# Autodesk Inventor assembly: Additional_Building
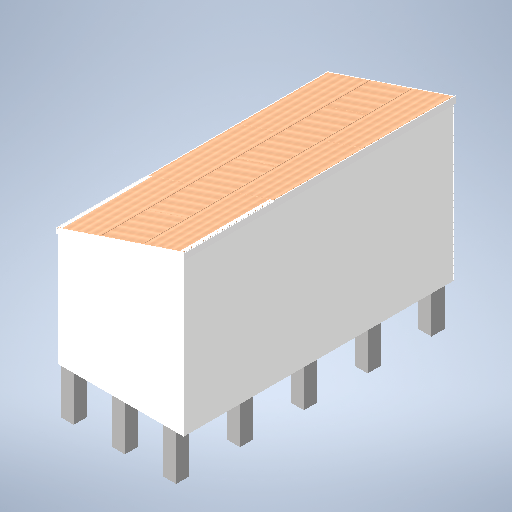
[picture p0: Inventor's stored thumbnail of the model, 512x512]
Saved by Autodesk Inventor 2025.1 (Build 291241020, 241B)
## iProperties
Created: 2024-08-02
Part Number: Additional_Building
Document SubType Name: Assembly
Designer: Tom
Author: Tom
## Documents named in this file (49)
- C:\Users\Tom\Documents\Inventor\Mobility\Additional_Building\Additional_Building.iam
- C:\Users\Tom\Documents\Inventor\Mobility\Additional_Building\Grid_Of_Piers.iam
- C:\Users\Tom\Documents\Inventor\Mobility\Additional_Building\Floor_System.iam
- C:\Users\Tom\Documents\Inventor\Mobility\Additional_Building\Walls.iam
- C:\Users\Tom\Documents\Inventor\Mobility\Additional_Building\Truss.iam
- C:\Users\Tom\Documents\Inventor\Mobility\Additional_Building\OSB_For_Walls_With_Dimensions_48_x_96_Inches.ipt
- C:\Users\Tom\Documents\Inventor\Mobility\Additional_Building\OSB_For_Walls_With_Dimensions_48_x_48_Inches.ipt
- C:\Users\Tom\Documents\Inventor\Mobility\Additional_Building\OSB_For_Roof_With_Dimensions_96_x_48.ipt
- C:\Users\Tom\Documents\Inventor\Mobility\Additional_Building\OSB_For_Walls_With_Dimensions_25.5_x_96_Inches.ipt
- C:\Users\Tom\Documents\Inventor\Mobility\Additional_Building\Subfascia_With_Dimensions_4.023_x_13.75_Inches.ipt
- C:\Users\Tom\Documents\Inventor\Mobility\Additional_Building\Subfascia_With_Dimensions_4.023_x_14.5_Inches.ipt
- C:\Users\Tom\Documents\Inventor\Mobility\Additional_Building\DensGlass_With_Dimensions_36.5_x_48_Inches.ipt
- C:\Users\Tom\Documents\Inventor\Mobility\Additional_Building\DensGlass_With_Dimensions_48_x_96_Inches.ipt
- C:\Users\Tom\Documents\Inventor\Mobility\Additional_Building\DensGlass_With_Dimensions_48_x_84.5_Inches.ipt
- C:\Users\Tom\Documents\Inventor\Mobility\Additional_Building\DensGlass_With_Dimensions_60.75_x_12_Inches.ipt
- C:\Users\Tom\Documents\Inventor\Mobility\Additional_Building\DensGlass_With_Dimensions_36.5_x_25.5_Inches.ipt
- C:\Users\Tom\Documents\Inventor\Mobility\Additional_Building\DensGlass_With_Dimensions_25.5_x_96_Inches.ipt
- C:\Users\Tom\Documents\Inventor\Mobility\Additional_Building\Siding_For_Back_Wall.iam
- C:\Users\Tom\Documents\Inventor\Mobility\Additional_Building\Fascia_For_Back.ipt
- C:\Users\Tom\Documents\Inventor\Mobility\Additional_Building\OSB_For_Side_And_Back.ipt
- C:\Users\Tom\Documents\Inventor\Mobility\Additional_Building\OSB_For_Roof_With_Dimensions_48_x_48.ipt
- C:\Users\Tom\Documents\Inventor\Mobility\Additional_Building\OSB_For_Roof_With_Dimensions_46.791_x_96.ipt
- C:\Users\Tom\Documents\Inventor\Mobility\Additional_Building\Stud_Between_Top_Plate_And_Rafter_1.ipt
- C:\Users\Tom\Documents\Inventor\Mobility\Additional_Building\Stud_Between_Top_Plate_And_Rafter_2.ipt
- C:\Users\Tom\Documents\Inventor\Mobility\Additional_Building\Stud_Between_Top_Plate_And_Rafter_3.ipt
- C:\Users\Tom\Documents\Inventor\Mobility\Additional_Building\Stud_Between_Top_Plate_And_Rafter_4.ipt
- C:\Users\Tom\Documents\Inventor\Mobility\Additional_Building\Stud_Between_Top_Plate_And_Rafter_5.ipt
- C:\Users\Tom\Documents\Inventor\Mobility\Additional_Building\Stud_Between_Top_Plate_And_Rafter_6.ipt
- C:\Users\Tom\Documents\Inventor\Mobility\Additional_Building\Stud_Between_Top_Plate_And_Rafter_7.ipt
- C:\Users\Tom\Documents\Inventor\Mobility\Additional_Building\Stud_Between_Top_Plate_And_Rafter_8.ipt
- C:\Users\Tom\Documents\Inventor\Mobility\Additional_Building\Stud_Between_Top_Plate_And_Rafter_9.ipt
- C:\Users\Tom\Documents\Inventor\Mobility\Additional_Building\Stud_With_Height_41.707_Inches.ipt
- C:\Users\Tom\Documents\Inventor\Mobility\Additional_Building\Support_For_Ceiling.ipt
- C:\Users\Tom\Documents\Inventor\Mobility\Additional_Building\OSB_For_Side_And_Front.ipt
- C:\Users\Tom\Documents\Inventor\Mobility\Additional_Building\OSB_For_Side_And_Top.ipt
- C:\Users\Tom\Documents\Inventor\Mobility\Additional_Building\Subfascia_With_Dimensions_5.798_x_13.75_Inches.ipt
- C:\Users\Tom\Documents\Inventor\Mobility\Additional_Building\Subfascia_With_Dimensions_5.798_x_14.5_Inches.ipt
- C:\Users\Tom\Documents\Inventor\Mobility\Additional_Building\OSB_For_Walls_With_Dimensions_20.604_x_48_Inches.ipt
- C:\Users\Tom\Documents\Inventor\Mobility\Additional_Building\OSB_For_Walls_With_Dimensions_20.604_x_96_Inches.ipt
- C:\Users\Tom\Documents\Inventor\Mobility\Additional_Building\Siding_For_Front_Wall.iam
- C:\Users\Tom\Documents\Inventor\Mobility\Additional_Building\Fascia_For_Front.ipt
- C:\Users\Tom\Documents\Inventor\Mobility\Additional_Building\OSB_For_Walls_With_Dimensions_48_x_85_Inches.ipt
- C:\Users\Tom\Documents\Inventor\Mobility\Additional_Building\OSB_For_Walls_With_Dimensions_37_x_48_Inches.ipt
- C:\Users\Tom\Documents\Inventor\Mobility\Additional_Building\Fascia_For_Side.ipt
- C:\Users\Tom\Documents\Inventor\Mobility\Additional_Building\Drip_Edge_For_Back.ipt
- C:\Users\Tom\Documents\Inventor\Mobility\Additional_Building\OSB_For_Rear_Roof.ipt
- C:\Users\Tom\Documents\Inventor\Mobility\Additional_Building\Siding_For_Left_Wall.iam
- C:\Users\Tom\Documents\Inventor\Mobility\Additional_Building\Siding_For_Right_Wall.iam
- C:\Users\Tom\Documents\Inventor\Mobility\Additional_Building\Drip_Edge_For_Front.ipt
## Components (175 placed, 48 different names)
1. Grid_Of_Piers:1 [sub-assembly] — Mate:1, Flush:1, Mate:2
2. Floor_System:1 [sub-assembly] — Mate:1, Flush:1, Mate:2, Mate:3, Flush:2, Flush:3, Flush:15, Flush:16, Flush:29, Flush:30, Flush:31, Flush:33
3. Walls:1 [sub-assembly] — Mate:3, Flush:2, Flush:3, Flush:4, Flush:5, Mate:4, Flush:7, Mate:5, Mate:9, Mate:10, Flush:17, Mate:12, Mate:15, Mate:18, Mate:68, Flush:48, Flush:49, Mate:69, Flush:50, Flush:51, Mate:70, Flush:52, Flush:53, Mate:71, Flush:54, Flush:55, Mate:72, Flush:56, Flush:57, Mate:73, Flush:58, Flush:59, Mate:74, Flush:60, Flush:61, Mate:75, Flush:62, Flush:63, Mate:76, Flush:64, Mate:78, Mate:90, Mate:113, Mate:116, Mate:119, Mate:121
4. Subfascia_With_Dimensions_4.023_x_13.75_Inches:1 — Mate:21, Flush:22, Flush:23
5. Subfascia_With_Dimensions_4.023_x_13.75_Inches:2 — Flush:26, Mate:23, Flush:27, Flush:39
6. DensGlass_With_Dimensions_36.5_x_48_Inches:1 — Mate:24, Flush:28, Flush:29, Mate:26
7. DensGlass_With_Dimensions_36.5_x_48_Inches:2 — Mate:27, Mate:28, Flush:31
8. DensGlass_With_Dimensions_48_x_84.5_Inches:1 — Mate:29, Flush:32, Mate:30, Mate:32, Mate:38, Mate:41, Mate:44
9. DensGlass_With_Dimensions_48_x_96_Inches:3 — Mate:31, Mate:32, Mate:33, Mate:35
10. DensGlass_With_Dimensions_48_x_84.5_Inches:2 — Mate:34, Mate:35, Mate:36, Mate:47
11. DensGlass_With_Dimensions_36.5_x_25.5_Inches:1 — Mate:39, Mate:40, Mate:41, Mate:43
12. DensGlass_With_Dimensions_36.5_x_25.5_Inches:2 — Mate:45, Mate:46, Mate:47
13. Siding_For_Back_Wall:1 [sub-assembly] — Mate:48, Flush:34, Flush:35
14. Siding_For_Front_Wall:1 [sub-assembly] — Flush:93, Flush:94, Mate:108
15. Fascia_For_Side:1 — Mate:126, Flush:103, Flush:105, Flush:108
16. Fascia_For_Side:2 — Mate:127, Flush:107, Flush:108
17. Drip_Edge_For_Back:1 — Flush:109, Mate:128, Mate:137
18. Siding_For_Left_Wall:1 [sub-assembly] — Mate:133, Flush:117, Mate:134
19. Siding_For_Right_Wall:1 [sub-assembly] — Mate:135, Mate:136, Flush:118
20. Drip_Edge_For_Front:1 — Mate:138, Flush:119, Mate:139
21. Truss:1 [sub-assembly] — Flush:6, Mate:23, Flush:27, Mate:50, Mate:56, Mate:77, Mate:79, Flush:65, Flush:67, Flush:69, Flush:71, Flush:73, Flush:75, Flush:77, Flush:79, Flush:81, Mate:92, Mate:96, Mate:109, Flush:103, Flush:104, Flush:115, Mate:132, Flush:116
22. Truss:2 [sub-assembly] — Flush:4, Flush:5, Mate:4, Mate:20, Mate:62, Mate:66, Mate:101, Flush:91, Mate:103, Flush:92
23. Truss:3 [sub-assembly] — Flush:6, Flush:7, Mate:5, Flush:26, Mate:81, Mate:82, Mate:83, Mate:84, Mate:85, Mate:86, Mate:87, Mate:88, Mate:89, Mate:91, Flush:82, Mate:99, Flush:87, Flush:88
24. Truss:4 [sub-assembly] — Mate:100, Flush:89, Flush:90
25. Truss:5 [sub-assembly]
26. Truss:6 [sub-assembly]
27. Truss:7 [sub-assembly]
28. Truss:8 [sub-assembly]
29. Truss:9 [sub-assembly]
30. Truss:10 [sub-assembly]
31. Truss:11 [sub-assembly]
32. Truss:12 [sub-assembly]
33. Truss:13 [sub-assembly]
34. Truss:14 [sub-assembly]
35. Truss:15 [sub-assembly] — Mate:63
36. Truss:16 [sub-assembly] — Mate:105
37. Truss:17 [sub-assembly]
38. Truss:18 [sub-assembly] — Mate:22, Flush:25
39. Truss:19 [sub-assembly] — Mate:21, Flush:22, Flush:23, Flush:24
40. OSB_For_Roof_With_Dimensions_96_x_48:4 — Mate:63, Mate:65
41. OSB_For_Roof_With_Dimensions_96_x_48:5
42. Subfascia_With_Dimensions_4.023_x_14.5_Inches:1 — Flush:24, Mate:22, Flush:25
43. Subfascia_With_Dimensions_4.023_x_14.5_Inches:2
44. Subfascia_With_Dimensions_4.023_x_14.5_Inches:3
45. Subfascia_With_Dimensions_4.023_x_14.5_Inches:4
46. Subfascia_With_Dimensions_4.023_x_14.5_Inches:5
47. Subfascia_With_Dimensions_4.023_x_14.5_Inches:6
48. Subfascia_With_Dimensions_4.023_x_14.5_Inches:7
49. Subfascia_With_Dimensions_4.023_x_14.5_Inches:8
50. Subfascia_With_Dimensions_4.023_x_14.5_Inches:9
51. Subfascia_With_Dimensions_4.023_x_14.5_Inches:10
52. Subfascia_With_Dimensions_4.023_x_14.5_Inches:11
53. Subfascia_With_Dimensions_4.023_x_14.5_Inches:12
54. Subfascia_With_Dimensions_4.023_x_14.5_Inches:13
55. Subfascia_With_Dimensions_4.023_x_14.5_Inches:14
56. Subfascia_With_Dimensions_4.023_x_14.5_Inches:15
57. Subfascia_With_Dimensions_4.023_x_14.5_Inches:16
58. DensGlass_With_Dimensions_48_x_96_Inches:1 — Mate:25, Mate:26, Flush:30, Mate:30, Mate:33
59. DensGlass_With_Dimensions_48_x_96_Inches:2 — Mate:28, Mate:36
60. DensGlass_With_Dimensions_60.75_x_12_Inches:1 — Mate:37, Mate:38, Flush:33
61. DensGlass_With_Dimensions_60.75_x_12_Inches:2 — Mate:48, Flush:34, Flush:35
62. DensGlass_With_Dimensions_60.75_x_12_Inches:3 — Mate:40
63. DensGlass_With_Dimensions_60.75_x_12_Inches:4 — Mate:57, Mate:115
64. DensGlass_With_Dimensions_25.5_x_96_Inches:1 — Mate:42, Mate:43, Mate:44
65. DensGlass_With_Dimensions_25.5_x_96_Inches:2 — Mate:46
66. Stud_Between_Top_Plate_And_Rafter_1:1 — Mate:68, Flush:48, Flush:49, Flush:66
67. Stud_Between_Top_Plate_And_Rafter_2:1 — Mate:69, Flush:50, Flush:51, Flush:68
68. Stud_Between_Top_Plate_And_Rafter_3:1 — Mate:70, Flush:52, Flush:53, Flush:70
69. Stud_Between_Top_Plate_And_Rafter_4:1 — Mate:71, Flush:54, Flush:55, Flush:72
70. Stud_Between_Top_Plate_And_Rafter_5:1 — Mate:72, Flush:56, Flush:57, Flush:74
71. Stud_Between_Top_Plate_And_Rafter_6:1 — Mate:73, Flush:58, Flush:59, Flush:76
72. Stud_Between_Top_Plate_And_Rafter_7:1 — Mate:74, Flush:60, Flush:61, Flush:78
73. Stud_Between_Top_Plate_And_Rafter_9:1 — Mate:76, Mate:77, Flush:64, Mate:80
74. Stud_Between_Top_Plate_And_Rafter_8:1 — Mate:75, Flush:62, Flush:63, Flush:80
75. Stud_Between_Top_Plate_And_Rafter_1:2
76. Stud_Between_Top_Plate_And_Rafter_2:2
77. Stud_Between_Top_Plate_And_Rafter_3:2
78. Stud_Between_Top_Plate_And_Rafter_4:2
79. Stud_Between_Top_Plate_And_Rafter_5:2
80. Stud_Between_Top_Plate_And_Rafter_6:2
81. Stud_Between_Top_Plate_And_Rafter_7:2
82. Stud_Between_Top_Plate_And_Rafter_9:2
83. Stud_Between_Top_Plate_And_Rafter_8:2
84. Stud_With_Height_41.707_Inches:1 — Mate:78, Mate:79, Mate:80
85. Stud_With_Height_41.707_Inches:2
86. Support_For_Ceiling:9 — Mate:89, Flush:81, Mate:90
87. Support_For_Ceiling:1 — Mate:81, Flush:65, Flush:66
88. Support_For_Ceiling:2 — Mate:82, Flush:67, Flush:68
89. Support_For_Ceiling:3 — Mate:83, Flush:69, Flush:70
90. Support_For_Ceiling:4 — Mate:84, Flush:71, Flush:72
91. Support_For_Ceiling:5 — Mate:85, Flush:73, Flush:74
92. Support_For_Ceiling:6 — Mate:86, Flush:75, Flush:76
93. Support_For_Ceiling:7 — Mate:87, Flush:77, Flush:78
94. Support_For_Ceiling:8 — Mate:88, Flush:79, Flush:80
95. Support_For_Ceiling:10 — Mate:91, Flush:82, Mate:92
96. Support_For_Ceiling:11
97. Support_For_Ceiling:12
98. Support_For_Ceiling:13
99. Support_For_Ceiling:14
100. Support_For_Ceiling:15
101. Support_For_Ceiling:16
102. Support_For_Ceiling:17
103. Support_For_Ceiling:18
104. Support_For_Ceiling:19
105. Support_For_Ceiling:20
106. Subfascia_With_Dimensions_5.798_x_13.75_Inches:1 — Mate:99, Flush:87, Flush:88
107. Subfascia_With_Dimensions_5.798_x_13.75_Inches:2
108. Subfascia_With_Dimensions_5.798_x_14.5_Inches:1 — Mate:100, Flush:89, Flush:90
109. Subfascia_With_Dimensions_5.798_x_14.5_Inches:2
110. Subfascia_With_Dimensions_5.798_x_14.5_Inches:3
111. Subfascia_With_Dimensions_5.798_x_14.5_Inches:4
112. Subfascia_With_Dimensions_5.798_x_14.5_Inches:5
113. Subfascia_With_Dimensions_5.798_x_14.5_Inches:6
114. Subfascia_With_Dimensions_5.798_x_14.5_Inches:7
115. Subfascia_With_Dimensions_5.798_x_14.5_Inches:8
116. Subfascia_With_Dimensions_5.798_x_14.5_Inches:9
117. Subfascia_With_Dimensions_5.798_x_14.5_Inches:10
118. Subfascia_With_Dimensions_5.798_x_14.5_Inches:11
119. Subfascia_With_Dimensions_5.798_x_14.5_Inches:12
120. Subfascia_With_Dimensions_5.798_x_14.5_Inches:13
121. Subfascia_With_Dimensions_5.798_x_14.5_Inches:14
122. Subfascia_With_Dimensions_5.798_x_14.5_Inches:15
123. Subfascia_With_Dimensions_5.798_x_14.5_Inches:16
124. OSB_For_Walls_With_Dimensions_25.5_x_96_Inches:1 — Mate:18, Flush:18, Mate:20, Mate:39
125. OSB_For_Walls_With_Dimensions_25.5_x_96_Inches:2 — Mate:42
126. OSB_For_Walls_With_Dimensions_25.5_x_96_Inches:3 — Mate:45
127. OSB_For_Walls_With_Dimensions_48_x_48_Inches:2 — Mate:15, Mate:16, Mate:17, Mate:29, Flush:32
128. OSB_For_Walls_With_Dimensions_48_x_48_Inches:1 — Mate:10, Mate:11, Flush:17, Mate:13, Mate:34
129. OSB_For_Walls_With_Dimensions_48_x_48_Inches:3 — Mate:102
130. OSB_For_Walls_With_Dimensions_48_x_48_Inches:4
131. OSB_For_Walls_With_Dimensions_48_x_96_Inches:13 — Mate:101, Mate:102, Flush:91, Mate:104, Mate:108
132. OSB_For_Walls_With_Dimensions_48_x_96_Inches:14 — Mate:106
133. OSB_For_Walls_With_Dimensions_48_x_96_Inches:15
134. OSB_For_Walls_With_Dimensions_20.604_x_96_Inches:1 — Mate:105, Mate:106, Mate:107
135. OSB_For_Walls_With_Dimensions_20.604_x_96_Inches:2
136. OSB_For_Walls_With_Dimensions_20.604_x_48_Inches:1 — Mate:103, Mate:104, Flush:92, Mate:107
137. OSB_For_Walls_With_Dimensions_20.604_x_48_Inches:2
138. Fascia_For_Back:1 — Mate:50, Flush:39, Flush:104, Flush:105, Flush:109, Mate:128, Mate:134
139. Fascia_For_Back:2
140. Fascia_For_Back:3 — Mate:136
141. Fascia_For_Front:1 — Mate:109, Flush:95, Flush:96, Mate:126, Mate:138, Flush:119
142. Fascia_For_Front:2
143. Fascia_For_Front:3 — Mate:127, Flush:107
144. OSB_For_Walls_With_Dimensions_48_x_96_Inches:16 — Mate:119, Mate:120, Flush:98, Mate:131, Mate:133, Flush:117
145. OSB_For_Walls_With_Dimensions_37_x_48_Inches:1 — Mate:121, Mate:122, Mate:131
146. OSB_For_Walls_With_Dimensions_48_x_48_Inches:5 — Mate:113, Mate:114, Mate:115, Mate:117, Mate:120
147. OSB_For_Walls_With_Dimensions_48_x_85_Inches:1 — Mate:116, Mate:117, Mate:118, Mate:122
148. OSB_For_Side_And_Back:1 — Mate:56, Mate:57, Flush:83, Mate:98, Mate:111, Mate:112, Mate:114, Mate:118
149. OSB_For_Side_And_Front:1 — Flush:83, Mate:97, Mate:111, Mate:112, Flush:97
150. OSB_For_Side_And_Top:1 — Mate:96, Mate:97, Flush:95, Flush:96, Flush:97, Flush:114
151. OSB_For_Walls_With_Dimensions_48_x_96_Inches:17 — Mate:135
152. OSB_For_Walls_With_Dimensions_37_x_48_Inches:2 — Flush:118
153. OSB_For_Walls_With_Dimensions_48_x_48_Inches:6
154. OSB_For_Walls_With_Dimensions_48_x_85_Inches:2
155. OSB_For_Side_And_Back:2
156. OSB_For_Side_And_Front:2
157. OSB_For_Side_And_Top:2
158. OSB_For_Roof_With_Dimensions_46.791_x_96:1 — Mate:66, Mate:67, Flush:47
159. OSB_For_Roof_With_Dimensions_46.791_x_96:2
160. OSB_For_Roof_With_Dimensions_46.791_x_96:3 — Flush:114, Mate:139
161. OSB_For_Rear_Roof:1 — Flush:115, Mate:132, Flush:116
162. OSB_For_Rear_Roof:2 — Mate:137
163. OSB_For_Rear_Roof:3
164. OSB_For_Roof_With_Dimensions_48_x_48:1 — Mate:62, Mate:65, Mate:67, Flush:47
165. OSB_For_Roof_With_Dimensions_48_x_48:2
166. OSB_For_Walls_With_Dimensions_48_x_96_Inches:1 — Mate:9, Flush:15, Flush:16, Mate:11, Mate:16, Flush:18, Mate:24, Flush:28, Mate:25, Mate:37
167. OSB_For_Walls_With_Dimensions_48_x_96_Inches:2
168. OSB_For_Walls_With_Dimensions_48_x_96_Inches:3 — Mate:14, Mate:27, Flush:98
169. OSB_For_Walls_With_Dimensions_48_x_96_Inches:4 — Mate:12, Mate:13, Mate:14, Mate:31
170. OSB_For_Walls_With_Dimensions_48_x_96_Inches:5 — Mate:17
171. OSB_For_Walls_With_Dimensions_48_x_96_Inches:8 — Flush:93, Flush:94
172. OSB_For_Walls_With_Dimensions_48_x_96_Inches:9
173. OSB_For_Walls_With_Dimensions_48_x_96_Inches:10
174. OSB_For_Walls_With_Dimensions_48_x_96_Inches:11
175. OSB_For_Walls_With_Dimensions_48_x_96_Inches:12
## Component patterns: (2 elements, first: Truss:1), (17 elements, first: Truss:3), (2 elements, first: OSB_For_Roof_With_Dimensions_96_x_48:4), (16 elements, first: Subfascia_With_Dimensions_4.023_x_14.5_Inches:1), (2 elements, first: DensGlass_With_Dimensions_48_x_96_Inches:1), (4 elements, first: DensGlass_With_Dimensions_60.75_x_12_Inches:1), (2 elements, first: DensGlass_With_Dimensions_25.5_x_96_Inches:1), (2 elements, first: Stud_Between_Top_Plate_And_Rafter_1:1 + Stud_Between_Top_Plate_And_Rafter_2:1 + Stud_Between_Top_Plate_And_Rafter_3:1 + Stud_Between_Top_Plate_And_Rafter_4:1 + Stud_Between_Top_Plate_And_Rafter_5:1 + Stud_Between_Top_Plate_And_Rafter_6:1 + Stud_Between_Top_Plate_And_Rafter_7:1 + Stud_Between_Top_Plate_And_Rafter_9:1 + Stud_Between_Top_Plate_And_Rafter_8:1), (2 elements, first: Stud_With_Height_41.707_Inches:1), (2 elements, first: Support_For_Ceiling:9 + Support_For_Ceiling:1 + Support_For_Ceiling:2 + Support_For_Ceiling:3 + Support_For_Ceiling:4 + Support_For_Ceiling:5 + Support_For_Ceiling:6 + Support_For_Ceiling:7 + Support_For_Ceiling:8 + Support_For_Ceiling:10), (2 elements, first: Subfascia_With_Dimensions_5.798_x_13.75_Inches:1), (16 elements, first: Subfascia_With_Dimensions_5.798_x_14.5_Inches:1), (3 elements, first: OSB_For_Walls_With_Dimensions_25.5_x_96_Inches:1), (2 elements, first: OSB_For_Walls_With_Dimensions_48_x_48_Inches:2 + OSB_For_Walls_With_Dimensions_48_x_48_Inches:1), (3 elements, first: OSB_For_Walls_With_Dimensions_48_x_96_Inches:13), (2 elements, first: OSB_For_Walls_With_Dimensions_20.604_x_96_Inches:1), (2 elements, first: OSB_For_Walls_With_Dimensions_20.604_x_48_Inches:1), (3 elements, first: Fascia_For_Back:1), (3 elements, first: Fascia_For_Front:1), (2 elements, first: OSB_For_Walls_With_Dimensions_48_x_96_Inches:16 + OSB_For_Walls_With_Dimensions_37_x_48_Inches:1 + OSB_For_Walls_With_Dimensions_48_x_48_Inches:5 + OSB_For_Walls_With_Dimensions_48_x_85_Inches:1 + OSB_For_Side_And_Back:1 + OSB_For_Side_And_Front:1 + OSB_For_Side_And_Top:1), (3 elements, first: OSB_For_Roof_With_Dimensions_46.791_x_96:1), (3 elements, first: OSB_For_Rear_Roof:1), (2 elements, first: OSB_For_Roof_With_Dimensions_48_x_48:1), (3 elements, first: OSB_For_Walls_With_Dimensions_48_x_96_Inches:1), (2 elements, first: OSB_For_Walls_With_Dimensions_48_x_96_Inches:4), Component Pattern 3:2 (3 elements), Component Pattern 4:2 (2 elements)
## Relationships (203: Mate 115, Flush 87, Angle 1)
- Mate:1: Grid_Of_Piers:1 ↔ Floor_System:1
- Flush:1: Grid_Of_Piers:1 ↔ Floor_System:1
- Mate:2: Grid_Of_Piers:1 ↔ Floor_System:1
- Mate:3: Floor_System:1 ↔ Walls:1
- Flush:2: Floor_System:1 ↔ Walls:1
- Flush:3: Floor_System:1 ↔ Walls:1
- Flush:4: Walls:1 ↔ Truss:2
- Flush:5: Walls:1 ↔ Truss:2
- Mate:4: Walls:1 ↔ Truss:2
- Flush:6 (387.35 mm): Truss:1 ↔ Truss:3
- Flush:7: Walls:1 ↔ Truss:3
- Mate:5: Walls:1 ↔ Truss:3
- Mate:9: Walls:1 ↔ OSB_For_Walls_With_Dimensions_48_x_96_Inches:1
- Flush:15: Floor_System:1 ↔ OSB_For_Walls_With_Dimensions_48_x_96_Inches:1
- Flush:16: Floor_System:1 ↔ OSB_For_Walls_With_Dimensions_48_x_96_Inches:1
- Mate:10: Walls:1 ↔ OSB_For_Walls_With_Dimensions_48_x_48_Inches:1
- Mate:11: OSB_For_Walls_With_Dimensions_48_x_48_Inches:1 ↔ OSB_For_Walls_With_Dimensions_48_x_96_Inches:1
- Flush:17: Walls:1 ↔ OSB_For_Walls_With_Dimensions_48_x_48_Inches:1
- Mate:12: Walls:1 ↔ OSB_For_Walls_With_Dimensions_48_x_96_Inches:4
- Mate:13: OSB_For_Walls_With_Dimensions_48_x_48_Inches:1 ↔ OSB_For_Walls_With_Dimensions_48_x_96_Inches:4
- Mate:14: OSB_For_Walls_With_Dimensions_48_x_96_Inches:3 ↔ OSB_For_Walls_With_Dimensions_48_x_96_Inches:4
- Mate:15: Walls:1 ↔ OSB_For_Walls_With_Dimensions_48_x_48_Inches:2
- Mate:16: OSB_For_Walls_With_Dimensions_48_x_48_Inches:2 ↔ OSB_For_Walls_With_Dimensions_48_x_96_Inches:1
- Mate:17: OSB_For_Walls_With_Dimensions_48_x_48_Inches:2 ↔ OSB_For_Walls_With_Dimensions_48_x_96_Inches:5
- Mate:18: Walls:1 ↔ OSB_For_Walls_With_Dimensions_25.5_x_96_Inches:1
- Flush:18: OSB_For_Walls_With_Dimensions_25.5_x_96_Inches:1 ↔ OSB_For_Walls_With_Dimensions_48_x_96_Inches:1
- Mate:20: Truss:2 ↔ OSB_For_Walls_With_Dimensions_25.5_x_96_Inches:1
- Mate:21: Subfascia_With_Dimensions_4.023_x_13.75_Inches:1 ↔ Truss:19
- Flush:22: Subfascia_With_Dimensions_4.023_x_13.75_Inches:1 ↔ Truss:19
- Flush:23: Subfascia_With_Dimensions_4.023_x_13.75_Inches:1 ↔ Truss:19
- Flush:24: Truss:19 ↔ Subfascia_With_Dimensions_4.023_x_14.5_Inches:1
- Mate:22: Truss:18 ↔ Subfascia_With_Dimensions_4.023_x_14.5_Inches:1
- Flush:25: Truss:18 ↔ Subfascia_With_Dimensions_4.023_x_14.5_Inches:1
- Flush:26: Subfascia_With_Dimensions_4.023_x_13.75_Inches:2 ↔ Truss:3
- Mate:23: Subfascia_With_Dimensions_4.023_x_13.75_Inches:2 ↔ Truss:1
- Flush:27: Subfascia_With_Dimensions_4.023_x_13.75_Inches:2 ↔ Truss:1
- Mate:24: DensGlass_With_Dimensions_36.5_x_48_Inches:1 ↔ OSB_For_Walls_With_Dimensions_48_x_96_Inches:1
- Flush:28 (292.1 mm): DensGlass_With_Dimensions_36.5_x_48_Inches:1 ↔ OSB_For_Walls_With_Dimensions_48_x_96_Inches:1
- Flush:29: Floor_System:1 ↔ DensGlass_With_Dimensions_36.5_x_48_Inches:1
- Mate:25: DensGlass_With_Dimensions_48_x_96_Inches:1 ↔ OSB_For_Walls_With_Dimensions_48_x_96_Inches:1
- Mate:26: DensGlass_With_Dimensions_36.5_x_48_Inches:1 ↔ DensGlass_With_Dimensions_48_x_96_Inches:1
- Flush:30: Floor_System:1 ↔ DensGlass_With_Dimensions_48_x_96_Inches:1
- Mate:27: DensGlass_With_Dimensions_36.5_x_48_Inches:2 ↔ OSB_For_Walls_With_Dimensions_48_x_96_Inches:3
- Mate:28: DensGlass_With_Dimensions_36.5_x_48_Inches:2 ↔ DensGlass_With_Dimensions_48_x_96_Inches:2
- Flush:31: Floor_System:1 ↔ DensGlass_With_Dimensions_36.5_x_48_Inches:2
- Mate:29: DensGlass_With_Dimensions_48_x_84.5_Inches:1 ↔ OSB_For_Walls_With_Dimensions_48_x_48_Inches:2
- Flush:32 (292.1 mm): DensGlass_With_Dimensions_48_x_84.5_Inches:1 ↔ OSB_For_Walls_With_Dimensions_48_x_48_Inches:2
- Mate:30: DensGlass_With_Dimensions_48_x_84.5_Inches:1 ↔ DensGlass_With_Dimensions_48_x_96_Inches:1
- Mate:31: DensGlass_With_Dimensions_48_x_96_Inches:3 ↔ OSB_For_Walls_With_Dimensions_48_x_96_Inches:4
- Mate:32: DensGlass_With_Dimensions_48_x_84.5_Inches:1 ↔ DensGlass_With_Dimensions_48_x_96_Inches:3
- Mate:33: DensGlass_With_Dimensions_48_x_96_Inches:3 ↔ DensGlass_With_Dimensions_48_x_96_Inches:1
- Mate:34: DensGlass_With_Dimensions_48_x_84.5_Inches:2 ↔ OSB_For_Walls_With_Dimensions_48_x_48_Inches:1
- Mate:35: DensGlass_With_Dimensions_48_x_96_Inches:3 ↔ DensGlass_With_Dimensions_48_x_84.5_Inches:2
- Mate:36: DensGlass_With_Dimensions_48_x_84.5_Inches:2 ↔ DensGlass_With_Dimensions_48_x_96_Inches:2
- Mate:37: DensGlass_With_Dimensions_60.75_x_12_Inches:1 ↔ OSB_For_Walls_With_Dimensions_48_x_96_Inches:1
- Mate:38: DensGlass_With_Dimensions_48_x_84.5_Inches:1 ↔ DensGlass_With_Dimensions_60.75_x_12_Inches:1
- Flush:33: Floor_System:1 ↔ DensGlass_With_Dimensions_60.75_x_12_Inches:1
- Mate:39: DensGlass_With_Dimensions_36.5_x_25.5_Inches:1 ↔ OSB_For_Walls_With_Dimensions_25.5_x_96_Inches:1
- Mate:40: DensGlass_With_Dimensions_36.5_x_25.5_Inches:1 ↔ DensGlass_With_Dimensions_60.75_x_12_Inches:3
- Mate:41: DensGlass_With_Dimensions_48_x_84.5_Inches:1 ↔ DensGlass_With_Dimensions_36.5_x_25.5_Inches:1
- Mate:42: DensGlass_With_Dimensions_25.5_x_96_Inches:1 ↔ OSB_For_Walls_With_Dimensions_25.5_x_96_Inches:2
- Mate:43: DensGlass_With_Dimensions_36.5_x_25.5_Inches:1 ↔ DensGlass_With_Dimensions_25.5_x_96_Inches:1
- Mate:44: DensGlass_With_Dimensions_48_x_84.5_Inches:1 ↔ DensGlass_With_Dimensions_25.5_x_96_Inches:1
- Mate:45: DensGlass_With_Dimensions_36.5_x_25.5_Inches:2 ↔ OSB_For_Walls_With_Dimensions_25.5_x_96_Inches:3
- Mate:46: DensGlass_With_Dimensions_36.5_x_25.5_Inches:2 ↔ DensGlass_With_Dimensions_25.5_x_96_Inches:2
- Mate:47: DensGlass_With_Dimensions_48_x_84.5_Inches:2 ↔ DensGlass_With_Dimensions_36.5_x_25.5_Inches:2
- Mate:48: Siding_For_Back_Wall:1 ↔ DensGlass_With_Dimensions_60.75_x_12_Inches:2
- Flush:34: Siding_For_Back_Wall:1 ↔ DensGlass_With_Dimensions_60.75_x_12_Inches:2
- Flush:35: Siding_For_Back_Wall:1 ↔ DensGlass_With_Dimensions_60.75_x_12_Inches:2
- Mate:50: Truss:1 ↔ Fascia_For_Back:1
- Flush:39 (-29.3688 mm): Subfascia_With_Dimensions_4.023_x_13.75_Inches:2 ↔ Fascia_For_Back:1
- Mate:56: Truss:1 ↔ OSB_For_Side_And_Back:1
- Mate:57: DensGlass_With_Dimensions_60.75_x_12_Inches:4 ↔ OSB_For_Side_And_Back:1
- Mate:62: Truss:2 ↔ OSB_For_Roof_With_Dimensions_48_x_48:1
- Mate:63: Truss:15 ↔ OSB_For_Roof_With_Dimensions_96_x_48:4
- Mate:65: OSB_For_Roof_With_Dimensions_96_x_48:4 ↔ OSB_For_Roof_With_Dimensions_48_x_48:1
- Mate:66: Truss:2 ↔ OSB_For_Roof_With_Dimensions_46.791_x_96:1
- Mate:67: OSB_For_Roof_With_Dimensions_46.791_x_96:1 ↔ OSB_For_Roof_With_Dimensions_48_x_48:1
- Flush:47: OSB_For_Roof_With_Dimensions_46.791_x_96:1 ↔ OSB_For_Roof_With_Dimensions_48_x_48:1
- Mate:68: Walls:1 ↔ Stud_Between_Top_Plate_And_Rafter_1:1
- Flush:48: Walls:1 ↔ Stud_Between_Top_Plate_And_Rafter_1:1
- Flush:49: Walls:1 ↔ Stud_Between_Top_Plate_And_Rafter_1:1
- Mate:69: Walls:1 ↔ Stud_Between_Top_Plate_And_Rafter_2:1
- Flush:50: Walls:1 ↔ Stud_Between_Top_Plate_And_Rafter_2:1
- Flush:51: Walls:1 ↔ Stud_Between_Top_Plate_And_Rafter_2:1
- Mate:70: Walls:1 ↔ Stud_Between_Top_Plate_And_Rafter_3:1
- Flush:52: Walls:1 ↔ Stud_Between_Top_Plate_And_Rafter_3:1
- Flush:53: Walls:1 ↔ Stud_Between_Top_Plate_And_Rafter_3:1
- Mate:71: Walls:1 ↔ Stud_Between_Top_Plate_And_Rafter_4:1
- Flush:54: Walls:1 ↔ Stud_Between_Top_Plate_And_Rafter_4:1
- Flush:55: Walls:1 ↔ Stud_Between_Top_Plate_And_Rafter_4:1
- Mate:72: Walls:1 ↔ Stud_Between_Top_Plate_And_Rafter_5:1
- Flush:56: Walls:1 ↔ Stud_Between_Top_Plate_And_Rafter_5:1
- Flush:57: Walls:1 ↔ Stud_Between_Top_Plate_And_Rafter_5:1
- Mate:73: Walls:1 ↔ Stud_Between_Top_Plate_And_Rafter_6:1
- Flush:58: Walls:1 ↔ Stud_Between_Top_Plate_And_Rafter_6:1
- Flush:59: Walls:1 ↔ Stud_Between_Top_Plate_And_Rafter_6:1
- Mate:74: Walls:1 ↔ Stud_Between_Top_Plate_And_Rafter_7:1
- Flush:60: Walls:1 ↔ Stud_Between_Top_Plate_And_Rafter_7:1
- Flush:61: Walls:1 ↔ Stud_Between_Top_Plate_And_Rafter_7:1
- Mate:75: Walls:1 ↔ Stud_Between_Top_Plate_And_Rafter_8:1
- Flush:62: Walls:1 ↔ Stud_Between_Top_Plate_And_Rafter_8:1
- Flush:63: Walls:1 ↔ Stud_Between_Top_Plate_And_Rafter_8:1
- Mate:76: Walls:1 ↔ Stud_Between_Top_Plate_And_Rafter_9:1
- Mate:77: Truss:1 ↔ Stud_Between_Top_Plate_And_Rafter_9:1
- Flush:64: Walls:1 ↔ Stud_Between_Top_Plate_And_Rafter_9:1
- Mate:78: Walls:1 ↔ Stud_With_Height_41.707_Inches:1
- Mate:79: Truss:1 ↔ Stud_With_Height_41.707_Inches:1
- Mate:80: Stud_Between_Top_Plate_And_Rafter_9:1 ↔ Stud_With_Height_41.707_Inches:1
- Mate:81: Truss:3 ↔ Support_For_Ceiling:1
- Flush:65: Truss:1 ↔ Support_For_Ceiling:1
- Flush:66: Stud_Between_Top_Plate_And_Rafter_1:1 ↔ Support_For_Ceiling:1
- Mate:82: Truss:3 ↔ Support_For_Ceiling:2
- Flush:67: Truss:1 ↔ Support_For_Ceiling:2
- Flush:68: Stud_Between_Top_Plate_And_Rafter_2:1 ↔ Support_For_Ceiling:2
- Mate:83: Truss:3 ↔ Support_For_Ceiling:3
- Flush:69: Truss:1 ↔ Support_For_Ceiling:3
- Flush:70: Stud_Between_Top_Plate_And_Rafter_3:1 ↔ Support_For_Ceiling:3
- Mate:84: Truss:3 ↔ Support_For_Ceiling:4
- Flush:71: Truss:1 ↔ Support_For_Ceiling:4
- Flush:72: Stud_Between_Top_Plate_And_Rafter_4:1 ↔ Support_For_Ceiling:4
- Mate:85: Truss:3 ↔ Support_For_Ceiling:5
- Flush:73: Truss:1 ↔ Support_For_Ceiling:5
- Flush:74: Stud_Between_Top_Plate_And_Rafter_5:1 ↔ Support_For_Ceiling:5
- Mate:86: Truss:3 ↔ Support_For_Ceiling:6
- Flush:75: Truss:1 ↔ Support_For_Ceiling:6
- Flush:76: Stud_Between_Top_Plate_And_Rafter_6:1 ↔ Support_For_Ceiling:6
- Mate:87: Truss:3 ↔ Support_For_Ceiling:7
- Flush:77: Truss:1 ↔ Support_For_Ceiling:7
- Flush:78: Stud_Between_Top_Plate_And_Rafter_7:1 ↔ Support_For_Ceiling:7
- Mate:88: Truss:3 ↔ Support_For_Ceiling:8
- Flush:79: Truss:1 ↔ Support_For_Ceiling:8
- Flush:80: Stud_Between_Top_Plate_And_Rafter_8:1 ↔ Support_For_Ceiling:8
- Mate:89: Truss:3 ↔ Support_For_Ceiling:9
- Flush:81: Truss:1 ↔ Support_For_Ceiling:9
- Mate:90: Walls:1 ↔ Support_For_Ceiling:9
- Mate:91: Truss:3 ↔ Support_For_Ceiling:10
- Flush:82: Truss:3 ↔ Support_For_Ceiling:10
- Mate:92: Truss:1 ↔ Support_For_Ceiling:10
- Flush:83: OSB_For_Side_And_Back:1 ↔ OSB_For_Side_And_Front:1
- Mate:96: Truss:1 ↔ OSB_For_Side_And_Top:1
- Mate:97: OSB_For_Side_And_Front:1 ↔ OSB_For_Side_And_Top:1
- Mate:98: OSB_For_Side_And_Back:1
- Angle:1 (0 deg)
- Mate:99: Truss:3 ↔ Subfascia_With_Dimensions_5.798_x_13.75_Inches:1
- Flush:87: Truss:3 ↔ Subfascia_With_Dimensions_5.798_x_13.75_Inches:1
- Flush:88: Truss:3 ↔ Subfascia_With_Dimensions_5.798_x_13.75_Inches:1
- Mate:100: Truss:4 ↔ Subfascia_With_Dimensions_5.798_x_14.5_Inches:1
- Flush:89: Truss:4 ↔ Subfascia_With_Dimensions_5.798_x_14.5_Inches:1
- Flush:90: Truss:4 ↔ Subfascia_With_Dimensions_5.798_x_14.5_Inches:1
- Mate:101: Truss:2 ↔ OSB_For_Walls_With_Dimensions_48_x_96_Inches:13
- Mate:102: OSB_For_Walls_With_Dimensions_48_x_48_Inches:3 ↔ OSB_For_Walls_With_Dimensions_48_x_96_Inches:13
- Flush:91: Truss:2 ↔ OSB_For_Walls_With_Dimensions_48_x_96_Inches:13
- Mate:103: Truss:2 ↔ OSB_For_Walls_With_Dimensions_20.604_x_48_Inches:1
- Mate:104: OSB_For_Walls_With_Dimensions_48_x_96_Inches:13 ↔ OSB_For_Walls_With_Dimensions_20.604_x_48_Inches:1
- Flush:92: Truss:2 ↔ OSB_For_Walls_With_Dimensions_20.604_x_48_Inches:1
- Mate:105: Truss:16 ↔ OSB_For_Walls_With_Dimensions_20.604_x_96_Inches:1
- Mate:106: OSB_For_Walls_With_Dimensions_48_x_96_Inches:14 ↔ OSB_For_Walls_With_Dimensions_20.604_x_96_Inches:1
- Mate:107: OSB_For_Walls_With_Dimensions_20.604_x_96_Inches:1 ↔ OSB_For_Walls_With_Dimensions_20.604_x_48_Inches:1
- Flush:93 (-6.35 mm): Siding_For_Front_Wall:1 ↔ OSB_For_Walls_With_Dimensions_48_x_96_Inches:8
- Flush:94 (-12.7 mm): Siding_For_Front_Wall:1 ↔ OSB_For_Walls_With_Dimensions_48_x_96_Inches:8
- Mate:108: Siding_For_Front_Wall:1 ↔ OSB_For_Walls_With_Dimensions_48_x_96_Inches:13
- Mate:109: Truss:1 ↔ Fascia_For_Front:1
- Flush:95 (-20.6375 mm): Fascia_For_Front:1 ↔ OSB_For_Side_And_Top:1
- Flush:96 (-43.0276 mm): Fascia_For_Front:1 ↔ OSB_For_Side_And_Top:1
- Mate:111: OSB_For_Side_And_Back:1 ↔ OSB_For_Side_And_Front:1
- Mate:112: OSB_For_Side_And_Back:1 ↔ OSB_For_Side_And_Front:1
- Flush:97: OSB_For_Side_And_Front:1 ↔ OSB_For_Side_And_Top:1
- Mate:113: Walls:1 ↔ OSB_For_Walls_With_Dimensions_48_x_48_Inches:5
- Mate:114: OSB_For_Walls_With_Dimensions_48_x_48_Inches:5 ↔ OSB_For_Side_And_Back:1
- Mate:115: DensGlass_With_Dimensions_60.75_x_12_Inches:4 ↔ OSB_For_Walls_With_Dimensions_48_x_48_Inches:5
- Mate:116: Walls:1 ↔ OSB_For_Walls_With_Dimensions_48_x_85_Inches:1
- Mate:117: OSB_For_Walls_With_Dimensions_48_x_48_Inches:5 ↔ OSB_For_Walls_With_Dimensions_48_x_85_Inches:1
- Mate:118: OSB_For_Walls_With_Dimensions_48_x_85_Inches:1 ↔ OSB_For_Side_And_Back:1
- Mate:119: Walls:1 ↔ OSB_For_Walls_With_Dimensions_48_x_96_Inches:16
- Mate:120: OSB_For_Walls_With_Dimensions_48_x_96_Inches:16 ↔ OSB_For_Walls_With_Dimensions_48_x_48_Inches:5
- Flush:98: OSB_For_Walls_With_Dimensions_48_x_96_Inches:16 ↔ OSB_For_Walls_With_Dimensions_48_x_96_Inches:3
- Mate:121: Walls:1 ↔ OSB_For_Walls_With_Dimensions_37_x_48_Inches:1
- Mate:122: OSB_For_Walls_With_Dimensions_37_x_48_Inches:1 ↔ OSB_For_Walls_With_Dimensions_48_x_85_Inches:1
- Mate:126: Fascia_For_Side:1 ↔ Fascia_For_Front:1
- Flush:103: Fascia_For_Side:1 ↔ Truss:1
- Flush:104 (-55.7276 mm): Truss:1 ↔ Fascia_For_Back:1
- Flush:105: Fascia_For_Side:1 ↔ Fascia_For_Back:1
- Mate:127: Fascia_For_Side:2 ↔ Fascia_For_Front:3
- Flush:107: Fascia_For_Side:2 ↔ Fascia_For_Front:3
- Flush:108: Fascia_For_Side:1 ↔ Fascia_For_Side:2
- Flush:109: Drip_Edge_For_Back:1 ↔ Fascia_For_Back:1
- Mate:128: Drip_Edge_For_Back:1 ↔ Fascia_For_Back:1
- Mate:131: OSB_For_Walls_With_Dimensions_48_x_96_Inches:16 ↔ OSB_For_Walls_With_Dimensions_37_x_48_Inches:1
- Flush:114: OSB_For_Side_And_Top:1 ↔ OSB_For_Roof_With_Dimensions_46.791_x_96:3
- Flush:115: Truss:1 ↔ OSB_For_Rear_Roof:1
- Mate:132: Truss:1 ↔ OSB_For_Rear_Roof:1
- Flush:116: Truss:1 ↔ OSB_For_Rear_Roof:1
- Mate:133: Siding_For_Left_Wall:1 ↔ OSB_For_Walls_With_Dimensions_48_x_96_Inches:16
- Flush:117 (-6.35 mm): Siding_For_Left_Wall:1 ↔ OSB_For_Walls_With_Dimensions_48_x_96_Inches:16
- Mate:134: Siding_For_Left_Wall:1 ↔ Fascia_For_Back:1
- Mate:135: Siding_For_Right_Wall:1 ↔ OSB_For_Walls_With_Dimensions_48_x_96_Inches:17
- Mate:136: Siding_For_Right_Wall:1 ↔ Fascia_For_Back:3
- Flush:118 (-6.35 mm): Siding_For_Right_Wall:1 ↔ OSB_For_Walls_With_Dimensions_37_x_48_Inches:2
- Mate:137: Drip_Edge_For_Back:1 ↔ OSB_For_Rear_Roof:2
- Mate:138: Drip_Edge_For_Front:1 ↔ Fascia_For_Front:1
- Flush:119: Drip_Edge_For_Front:1 ↔ Fascia_For_Front:1
- Mate:139: Drip_Edge_For_Front:1 ↔ OSB_For_Roof_With_Dimensions_46.791_x_96:3
